# Autodesk Inventor assembly: 6P Sprocket
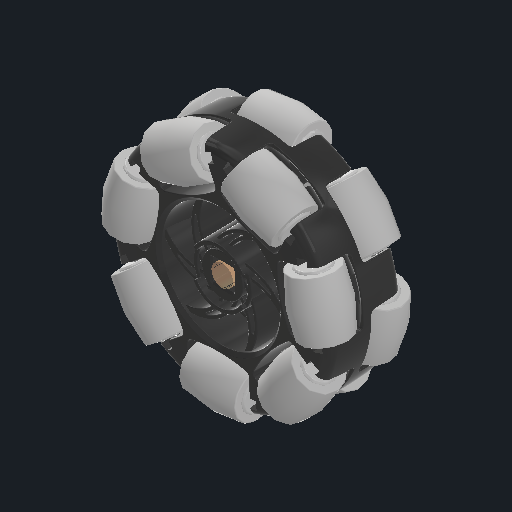
[picture p0: Inventor's stored thumbnail of the model, 512x512]
Saved by Autodesk Inventor 2024 (Build 280153000, 153)
## iProperties
Created: 2022-08-02
Part Number: 6P Sprocket
Document SubType Name: Assembly
Designer: ylu12
Author: ylu12
## Documents named in this file (27)
- \\Mac\Home\Desktop\code\1599V-VRC\Cad\Motion\Wheels\Omni Wheel.iam
- \\Mac\Home\Desktop\code\1599V-VRC\Cad\Motion\Wheels\Reference Files\2.75 Omni.ipt
- \\Mac\Home\Desktop\code\1599V-VRC\Cad\Motion\Wheels\Reference Files\2.75 Omni Antistatic.ipt
- \\Mac\Home\Desktop\code\1599V-VRC\Cad\Motion\Wheels\Reference Files\4 Omni.ipt
- \\Mac\Home\Desktop\code\1599V-VRC\Cad\Motion\Wheels\Reference Files\3.25 Omni.ipt
- \\Mac\Home\Desktop\code\1599V-VRC\Cad\Motion\Wheels\Reference Files\3.25 Omni Antistatic.ipt
- \\Mac\Home\Desktop\code\1599V-VRC\Cad\Motion\Wheels\Reference Files\4 Omni Antistatic.ipt
- \\Mac\Home\Desktop\code\1599V-VRC\Cad\Motion\Insert Circle.ipt
- \\Mac\Home\Desktop\code\1599V-VRC\Cad\Motion\Insert Square.ipt
- 2.75 Omni AS, Circle.iam
- 2.75 Omni AS, No Insert.iam
- 2.75 Omni AS, Square.iam
- 2.75 Omni, Circle.iam
- 2.75 Omni, No Insert.iam
- 2.75 Omni, Square.iam
- 3.25 Omni AS, Circle.iam
- 3.25 Omni AS, No Insert.iam
- 3.25 Omni AS, Square.iam
- 3.25 Omni, Circle.iam
- 3.25 Omni, No Insert.iam
- 3.25 Omni, Square.iam
- 4 Omni AS, Circle.iam
- 4 Omni AS, No Insert.iam
- 4 Omni AS, Square.iam
- 4 Omni, Circle.iam
- 4 Omni, No Insert.iam
- 4 Omni, Square.iam
## Components (10 placed, 10 different names)
1. 2.75 Omni
2. 2.75 Omni Antistatic
3. 3.25 Omni
4. 3.25 Omni Antistatic
5. 4 Omni Antistatic
6. 4 Omni — Mate:15, Mate:16, Flush:8
7. Circle 1 — Flush:12, Flush:13, Flush:14, Mate:20, Angle:2
8. Circle 2 — Flush:12, Flush:13, Mate:19
9. Square 1 — Mate:17, Flush:10, Flush:11
10. Square 2 — Flush:9, Flush:10, Flush:11, Mate:18, Angle:1
## Relationships (30: Mate 16, Flush 12, Angle 2)
- [Mate]: 2.75 Omni
- [Mate]: 2.75 Omni
- [Flush]: 2.75 Omni
- [Flush]: 2.75 Omni Antistatic
- [Flush]: 3.25 Omni
- [Flush]: 3.25 Omni Antistatic
- [Flush]: 4 Omni Antistatic
- [Mate]: 2.75 Omni Antistatic
- [Mate]: 2.75 Omni Antistatic
- [Mate]: 3.25 Omni
- [Mate]: 3.25 Omni
- [Mate]: 3.25 Omni Antistatic
- [Mate]: 3.25 Omni Antistatic
- [Mate]: 4 Omni Antistatic
- [Mate]: 4 Omni Antistatic
- Mate:15: 4 Omni
- Mate:16: 4 Omni
- Flush:8: 4 Omni
- Flush:9: Square 2
- Mate:17: Square 1
- Flush:10: Square 1 ↔ Square 2
- Flush:11: Square 1 ↔ Square 2
- Mate:18: Square 2
- Angle:1 (0 deg): Square 2
- Flush:12: Circle 1 ↔ Circle 2
- Flush:13: Circle 1 ↔ Circle 2
- Mate:19: Circle 2
- Flush:14: Circle 1
- Mate:20: Circle 1
- Angle:2 (0 deg): Circle 1
## Named parameters: HalfWheelWidth = 9.98 mm
